# Autodesk Inventor assembly: Hauptteil
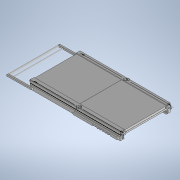
[picture p0: Inventor's stored thumbnail of the model, 180x180]
Saved by Autodesk Inventor 2020.3 (Build 243373000, 373)
## iProperties
Created: 2020-09-30
Part Number: Hauptteil
Document SubType Name: Assembly
Designer: Mara
Author: Mara
## Documents named in this file (10)
- C:\Users\Mara\Masterarbeit_CAD\Rampe\Hauptteil.iam
- C:\Users\Mara\Masterarbeit_CAD\Rampe\o_lange_Stange.ipt
- C:\Users\Mara\Masterarbeit_CAD\Rampe\u_lange_Stange.ipt
- C:\Users\Mara\Masterarbeit_CAD\Rampe\o_fache_Stange.ipt
- C:\Users\Mara\Masterarbeit_CAD\Rampe\o_grosses_Brett.ipt
- C:\Users\Mara\Masterarbeit_CAD\Rampe\o_Einlegplatten.ipt
- C:\Users\Mara\Masterarbeit_CAD\Rampe\u_g_Hoehenverstellung.ipt
- C:\Users\Mara\Masterarbeit_CAD\Rampe\u_k_Hoehenverstellung.ipt
- C:\Users\Mara\Masterarbeit_CAD\Rampe\u_lange_Stange_MIR.ipt
- C:\Users\Mara\Masterarbeit_CAD\Rampe\o_Plattenstopper.ipt
## Components (15 placed, 9 different names)
1. o_lange_Stange:1 — Mate:2, Flush:3, Flush:4, Mate:4, Flush:5, Flush:6, Mate:9, Mate:10, Flush:15, Rotational:4, Rotational:5
2. o_fache_Stange:1 — Mate:3, Flush:7, Flush:8
3. o_grosses_Brett:1 — Mate:1, Flush:1, Flush:2, Mate:2, Flush:3, Flush:4, Mate:7, Mate:8, Mate:12, Flush:16, Mate:13, Flush:17, Flush:18
4. o_fache_Stange:2 — Mate:4, Flush:5, Flush:6
5. o_lange_Stange:2 — Mate:1, Flush:1, Flush:2, Mate:3, Flush:7, Flush:8, Rotational:3, Rotational:6
6. u_lange_Stange:2 — Mate:12, Flush:15, Flush:16, Rotational:1, Rotational:2
7. o_Einlegplatten:1 — Mate:7, Mate:9
8. o_Einlegplatten:2 — Mate:8, Mate:10
9. u_g_Hoehenverstellung:1 — Rotational:1
10. u_k_Hoehenverstellung:1 — Rotational:2
11. u_lange_Stange_MIR:1 — Mate:13, Flush:17, Flush:18
12. o_Plattenstopper:1 — Rotational:3
13. o_Plattenstopper:2 — Rotational:4
14. o_Plattenstopper:3 — Rotational:6
15. o_Plattenstopper:4 — Rotational:5
## Relationships (28: Flush 12, Mate 10, RevoluteJoint 6)
- Mate:1: o_grosses_Brett:1 ↔ o_lange_Stange:2
- Flush:1: o_grosses_Brett:1 ↔ o_lange_Stange:2
- Flush:2: o_grosses_Brett:1 ↔ o_lange_Stange:2
- Mate:2: o_lange_Stange:1 ↔ o_grosses_Brett:1
- Flush:3: o_lange_Stange:1 ↔ o_grosses_Brett:1
- Flush:4: o_lange_Stange:1 ↔ o_grosses_Brett:1
- Mate:3: o_fache_Stange:1 ↔ o_lange_Stange:2
- Mate:4: o_lange_Stange:1 ↔ o_fache_Stange:2
- Flush:5: o_lange_Stange:1 ↔ o_fache_Stange:2
- Flush:6: o_lange_Stange:1 ↔ o_fache_Stange:2
- Flush:7: o_fache_Stange:1 ↔ o_lange_Stange:2
- Flush:8: o_fache_Stange:1 ↔ o_lange_Stange:2
- Mate:7: o_grosses_Brett:1 ↔ o_Einlegplatten:1
- Mate:8: o_grosses_Brett:1 ↔ o_Einlegplatten:2
- Mate:9 (2 mm): o_lange_Stange:1 ↔ o_Einlegplatten:1
- Mate:10 (2 mm): o_lange_Stange:1 ↔ o_Einlegplatten:2
- Mate:12: o_grosses_Brett:1 ↔ u_lange_Stange:2
- Flush:15: o_lange_Stange:1 ↔ u_lange_Stange:2
- Flush:16: o_grosses_Brett:1 ↔ u_lange_Stange:2
- Rotational:1 [RevoluteJoint] (2 mm): u_lange_Stange:2 ↔ u_g_Hoehenverstellung:1
- Rotational:2 [RevoluteJoint] (2 mm): u_lange_Stange:2 ↔ u_k_Hoehenverstellung:1
- Mate:13: o_grosses_Brett:1 ↔ u_lange_Stange_MIR:1
- Flush:17: o_grosses_Brett:1 ↔ u_lange_Stange_MIR:1
- Flush:18: o_grosses_Brett:1 ↔ u_lange_Stange_MIR:1
- Rotational:3 [RevoluteJoint]: o_lange_Stange:2 ↔ o_Plattenstopper:1
- Rotational:4 [RevoluteJoint]: o_lange_Stange:1 ↔ o_Plattenstopper:2
- Rotational:5 [RevoluteJoint]: o_lange_Stange:1 ↔ o_Plattenstopper:4
- Rotational:6 [RevoluteJoint]: o_lange_Stange:2 ↔ o_Plattenstopper:3
